# Autodesk Inventor assembly: BP_BOX2
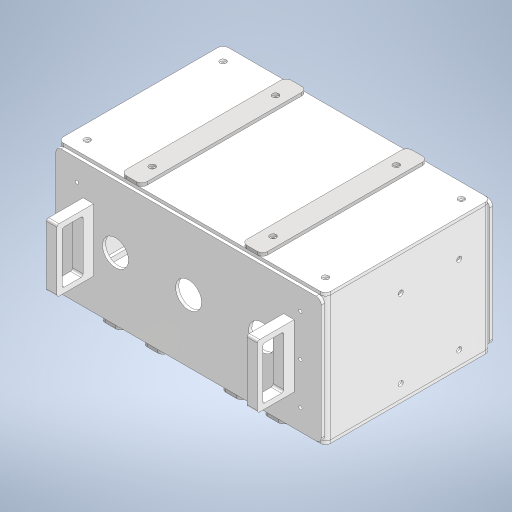
[picture p0: Inventor's stored thumbnail of the model, 512x512]
Saved by Autodesk Inventor 2024.3 (Build 283343000, 343)
## iProperties
Created: 2025-10-31
Part Number: BP_BOX2
Document SubType Name: Assembly
Designer: 佐藤智貴
Author: 佐藤智貴
## Documents named in this file (9)
- C:\Users\佐藤智貴\OneDrive - Chiba Institute of Technology\ドキュメント\Inventor\Biped_Robot2\BP_BOX2.iam
- C:\Users\佐藤智貴\OneDrive - Chiba Institute of Technology\ドキュメント\Inventor\Biped_Robot2\BP_BOX-handle.ipt
- C:\Users\佐藤智貴\OneDrive - Chiba Institute of Technology\ドキュメント\Inventor\Biped_Robot2\BP_BOX-Above.ipt
- C:\Users\佐藤智貴\OneDrive - Chiba Institute of Technology\ドキュメント\Inventor\Biped_Robot2\BP_BOX-Under.ipt
- C:\Users\佐藤智貴\OneDrive - Chiba Institute of Technology\ドキュメント\Inventor\Biped_Robot2\BP_BOX-Bar.ipt
- C:\Users\佐藤智貴\OneDrive - Chiba Institute of Technology\ドキュメント\Inventor\Biped_Robot2\BP_BOX-Side-120.ipt
- C:\Users\佐藤智貴\OneDrive - Chiba Institute of Technology\ドキュメント\Inventor\Biped_Robot2\BP_BOX-Front-120.ipt
- C:\Users\佐藤智貴\OneDrive - Chiba Institute of Technology\ドキュメント\Inventor\Biped_Robot2\BP_BOX-Back-120.ipt
- C:\Users\佐藤智貴\OneDrive - Chiba Institute of Technology\ドキュメント\Inventor\Biped_Robot2\BP_BOX-Side-120-2.ipt
## Components (14 placed, 8 different names)
1. BP_BOX-Above:1 — 挿入:16, 挿入:17, 挿入:18, 挿入:19, 挿入:43, 挿入:46
2. BP_BOX-handle:1 — 挿入:36, 挿入:37
3. BP_BOX-handle:2 — 挿入:38, 挿入:39
4. BP_BOX-Under:1 — 挿入:20, 挿入:21, 挿入:22, 挿入:23, 挿入:24, 挿入:25, 挿入:26, 挿入:27, 挿入:42, 挿入:45, 挿入:47
5. BP_BOX-Bar:1 — 挿入:16, 挿入:17
6. BP_BOX-Bar:2 — 挿入:18, 挿入:19
7. BP_BOX-Bar:3 — 挿入:21, 挿入:26
8. BP_BOX-Bar:4 — 挿入:22, 挿入:25
9. BP_BOX-Bar:5 — 挿入:23, 挿入:24
10. BP_BOX-Bar:6 — 挿入:20, 挿入:27
11. BP_BOX-Front-120:1 — 挿入:36, 挿入:37, 挿入:38, 挿入:39, 挿入:44, 挿入:49
12. BP_BOX-Back-120:1 — 挿入:48
13. BP_BOX-Side-120:3 — 挿入:42, 挿入:43, 挿入:44, 挿入:45
14. BP_BOX-Side-120-2:1 — 挿入:46, 挿入:47, 挿入:48, 挿入:49
## Relationships (24: Insert 24)
- 挿入:16 [Insert]: BP_BOX-Above:1 ↔ BP_BOX-Bar:1
- 挿入:17 [Insert]: BP_BOX-Above:1 ↔ BP_BOX-Bar:1
- 挿入:18 [Insert]: BP_BOX-Above:1 ↔ BP_BOX-Bar:2
- 挿入:19 [Insert]: BP_BOX-Above:1 ↔ BP_BOX-Bar:2
- 挿入:20 [Insert]: BP_BOX-Under:1 ↔ BP_BOX-Bar:6
- 挿入:21 [Insert]: BP_BOX-Under:1 ↔ BP_BOX-Bar:3
- 挿入:22 [Insert]: BP_BOX-Under:1 ↔ BP_BOX-Bar:4
- 挿入:23 [Insert]: BP_BOX-Under:1 ↔ BP_BOX-Bar:5
- 挿入:24 [Insert]: BP_BOX-Under:1 ↔ BP_BOX-Bar:5
- 挿入:25 [Insert]: BP_BOX-Under:1 ↔ BP_BOX-Bar:4
- 挿入:26 [Insert]: BP_BOX-Under:1 ↔ BP_BOX-Bar:3
- 挿入:27 [Insert]: BP_BOX-Under:1 ↔ BP_BOX-Bar:6
- 挿入:36 [Insert]: BP_BOX-handle:1 ↔ BP_BOX-Front-120:1
- 挿入:37 [Insert]: BP_BOX-handle:1 ↔ BP_BOX-Front-120:1
- 挿入:38 [Insert]: BP_BOX-handle:2 ↔ BP_BOX-Front-120:1
- 挿入:39 [Insert]: BP_BOX-handle:2 ↔ BP_BOX-Front-120:1
- 挿入:42 [Insert]: BP_BOX-Under:1 ↔ BP_BOX-Side-120:3
- 挿入:43 [Insert]: BP_BOX-Above:1 ↔ BP_BOX-Side-120:3
- 挿入:44 [Insert]: BP_BOX-Front-120:1 ↔ BP_BOX-Side-120:3
- 挿入:45 [Insert]: BP_BOX-Under:1 ↔ BP_BOX-Side-120:3
- 挿入:46 [Insert]: BP_BOX-Above:1 ↔ BP_BOX-Side-120-2:1
- 挿入:47 [Insert]: BP_BOX-Under:1 ↔ BP_BOX-Side-120-2:1
- 挿入:48 [Insert]: BP_BOX-Back-120:1 ↔ BP_BOX-Side-120-2:1
- 挿入:49 [Insert]: BP_BOX-Front-120:1 ↔ BP_BOX-Side-120-2:1
